# Autodesk Inventor assembly: non integrated hatch
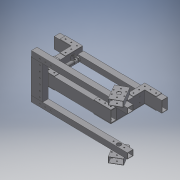
[picture p0: Inventor's stored thumbnail of the model, 180x180]
Saved by Autodesk Inventor 2018 (Build 220112000, 112)
## iProperties
Created: 2019-01-26
Part Number: non integrated hatch
Document SubType Name: Assembly
Designer: s-4008082
Author: s-4008082
## Documents named in this file (10)
- C:\Users\s-4008082\Downloads\2019CAD-master\2019CAD-master\Hatch design with heightened hatch\non integrated hatch.iam
- C:\Users\s-4008082\Downloads\2019CAD-master\2019CAD-master\Hatch design with heightened hatch\left arm.ipt
- C:\Users\s-4008082\Downloads\2019CAD-master\2019CAD-master\Hatch design with heightened hatch\push bar.ipt
- C:\Users\s-4008082\Downloads\2019CAD-master\2019CAD-master\Hatch design with heightened hatch\PARTserver02019011803125824465437192d056f\AIS2018\021-DXP(F,D-770).iam
- C:\Users\s-4008082\Downloads\2019CAD-master\2019CAD-master\Hatch design with heightened hatch\Bracing 3x3.ipt
- C:\Users\s-4008082\Downloads\ATACHMENT BAR.ipt
- C:\Users\s-4008082\Downloads\2019CAD-master\2019CAD-master\Hatch design with heightened hatch\Mounting part.ipt
- C:\Users\s-4008082\Downloads\2019CAD-master\2019CAD-master\Hatch design with heightened hatch\mounting part 2.ipt
- C:\Users\s-4008082\Downloads\2019CAD-master\2019CAD-master\Hatch design with heightened hatch\bar thing.ipt
- C:\Users\s-4008082\Downloads\2019CAD-master\2019CAD-master\Hatch design with heightened hatch\hub attachment.ipt
## Components (21 placed, 9 different names)
1. left arm:1 — Flush:23, Flush:28, Flush:29, Flush:32, Mate:37, Flush:34, Mate:38, Flush:35, Mate:41, Mate:42, Flush:37, Mate:47
2. push bar:1
3. 021-DXP(F,D-770):1 [sub-assembly] — Mate:41, Mate:42, Flush:37, Mate:47, Flush:43, Flush:46, Flush:47
4. 021-DXP(F,D-770):2 [sub-assembly] — Flush:43, Mate:50, Flush:46, Flush:47
5. Bracing 3x3:1 — Flush:28, Flush:29, Flush:30, Mate:38
6. Bracing 3x3:2 — Flush:22, Flush:31, Flush:32, Flush:33, Mate:37
7. Bracing 3x3:3 — Mate:33
8. Bracing 3x3:4 — Mate:30, Flush:24
9. Bracing 3x3:5 — Mate:36
10. Bracing 3x3:6
11. Bracing 3x3:7 — Flush:45
12. Bracing 3x3:8 — Mate:39, Mate:40, Flush:36
13. ATACHMENT BAR:1 — Mate:36, Flush:35, Mate:39, Mate:40, Flush:36, Mate:43, Mate:44, Mate:48, Mate:49, Flush:44
14. Mounting part:1 — Mate:43, Mate:44, Mate:45, Flush:38, Flush:39, Mate:46, Flush:41, Flush:42, Mate:48
15. mounting part 2:1 — Mate:45, Flush:38, Flush:39, Mate:51, Mate:52, Mate:56
16. mounting part 2:2 — Mate:46, Flush:41, Flush:42, Mate:53, Mate:54, Mate:55
17. bar thing:1 — Flush:22, Flush:23, Flush:30, Flush:31, Flush:33, Flush:34
18. bar thing:2 — Mate:30, Flush:24, Mate:33
19. left arm:2 — Mate:49, Flush:44, Flush:45, Mate:50
20. hub attachment:1 — Mate:51, Mate:52, Mate:56
21. hub attachment:2 — Mate:53, Mate:54, Mate:55
## Relationships (59: Mate 35, Flush 24)
- [Flush]: left arm:1 ↔ Bracing 3x3:2
- [Mate] (2.54 mm): push bar:1 ↔ 021-DXP(F,D-770):2
- [Mate]: push bar:1 ↔ 021-DXP(F,D-770):2
- [Mate] (2.54 mm): push bar:1 ↔ 021-DXP(F,D-770):1
- [Mate]: push bar:1 ↔ 021-DXP(F,D-770):1
- [Flush]: left arm:1 ↔ ATACHMENT BAR:1
- [Mate]: left arm:1 ↔ ATACHMENT BAR:1
- [Mate]: Bracing 3x3:6 ↔ ATACHMENT BAR:1
- [Mate]: Bracing 3x3:6 ↔ ATACHMENT BAR:1
- [Mate]: left arm:1 ↔ Bracing 3x3:5
- [Mate]: Bracing 3x3:5 ↔ ATACHMENT BAR:1
- [Mate]: Bracing 3x3:5 ↔ ATACHMENT BAR:1
- [Mate]: Bracing 3x3:7 ↔ ATACHMENT BAR:1
- [Mate]: Bracing 3x3:7 ↔ ATACHMENT BAR:1
- Flush:22: Bracing 3x3:2 ↔ bar thing:1
- Flush:23: left arm:1 ↔ bar thing:1
- Mate:30: Bracing 3x3:4 ↔ bar thing:2
- Flush:24: Bracing 3x3:4 ↔ bar thing:2
- Mate:33: Bracing 3x3:3 ↔ bar thing:2
- Mate:36: Bracing 3x3:5 ↔ ATACHMENT BAR:1
- Flush:28: left arm:1 ↔ Bracing 3x3:1
- Flush:29: left arm:1 ↔ Bracing 3x3:1
- Flush:30: Bracing 3x3:1 ↔ bar thing:1
- Flush:31: Bracing 3x3:2 ↔ bar thing:1
- Flush:32: left arm:1 ↔ Bracing 3x3:2
- Flush:33: Bracing 3x3:2 ↔ bar thing:1
- Mate:37: left arm:1 ↔ Bracing 3x3:2
- Flush:34: left arm:1 ↔ bar thing:1
- Mate:38: left arm:1 ↔ Bracing 3x3:1
- Flush:35: left arm:1 ↔ ATACHMENT BAR:1
- Mate:39: Bracing 3x3:8 ↔ ATACHMENT BAR:1
- Mate:40: Bracing 3x3:8 ↔ ATACHMENT BAR:1
- Flush:36: Bracing 3x3:8 ↔ ATACHMENT BAR:1
- Mate:41: left arm:1 ↔ 021-DXP(F,D-770):1
- Mate:42: left arm:1 ↔ 021-DXP(F,D-770):1
- Flush:37 (38.1 mm): left arm:1 ↔ 021-DXP(F,D-770):1
- Mate:43: ATACHMENT BAR:1 ↔ Mounting part:1
- Mate:44 (-101.6 mm): ATACHMENT BAR:1 ↔ Mounting part:1
- Mate:45: Mounting part:1 ↔ mounting part 2:1
- Flush:38: Mounting part:1 ↔ mounting part 2:1
- Flush:39: Mounting part:1 ↔ mounting part 2:1
- Mate:46: Mounting part:1 ↔ mounting part 2:2
- Flush:41: Mounting part:1 ↔ mounting part 2:2
- Flush:42: Mounting part:1 ↔ mounting part 2:2
- Mate:47: left arm:1 ↔ 021-DXP(F,D-770):1
- Flush:43: 021-DXP(F,D-770):1 ↔ 021-DXP(F,D-770):2
- Mate:48: ATACHMENT BAR:1 ↔ Mounting part:1
- Mate:49: ATACHMENT BAR:1 ↔ left arm:2
- Flush:44: ATACHMENT BAR:1 ↔ left arm:2
- Flush:45: Bracing 3x3:7 ↔ left arm:2
- Mate:50: 021-DXP(F,D-770):2 ↔ left arm:2
- Flush:46: 021-DXP(F,D-770):1 ↔ 021-DXP(F,D-770):2
- Flush:47: 021-DXP(F,D-770):1 ↔ 021-DXP(F,D-770):2
- Mate:51: mounting part 2:1 ↔ hub attachment:1
- Mate:52: mounting part 2:1 ↔ hub attachment:1
- Mate:53: mounting part 2:2 ↔ hub attachment:2
- Mate:54: mounting part 2:2 ↔ hub attachment:2
- Mate:55: mounting part 2:2 ↔ hub attachment:2
- Mate:56: mounting part 2:1 ↔ hub attachment:1
